# Autodesk Inventor assembly: Montagem peças superiores
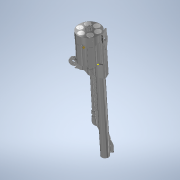
[picture p0: Inventor's stored thumbnail of the model, 180x180]
Saved by Autodesk Inventor 2021 (Build 250183000, 183)
## iProperties
Created: 2020-11-29
Part Number: Montagem peças superiores
Document SubType Name: Assembly
Designer: Bruno
Author: Bruno
## Documents named in this file (8)
- C:\Users\Bruno\Documents\Quadirmestre Suplementar\Projeto Assistido por Computador\Novas peças revólver\Montagem peças superiores.iam
- C:\Users\Bruno\Documents\Quadirmestre Suplementar\Projeto Assistido por Computador\Novas peças revólver\Cano do revólver.ipt
- C:\Users\Bruno\Documents\Quadirmestre Suplementar\Projeto Assistido por Computador\Novas peças revólver\Peça 15.ipt
- C:\Users\Bruno\Documents\Quadirmestre Suplementar\Projeto Assistido por Computador\Novas peças revólver\Peça 16.ipt
- C:\Users\Bruno\Documents\Quadirmestre Suplementar\Projeto Assistido por Computador\Novas peças revólver\Peça 17.ipt
- C:\Users\Bruno\Documents\Quadirmestre Suplementar\Projeto Assistido por Computador\Novas peças revólver\Baril do revólver.ipt
- C:\Users\Bruno\Documents\Quadirmestre Suplementar\Projeto Assistido por Computador\Novas peças revólver\Peça 18.ipt
- C:\Users\Bruno\Documents\Quadirmestre Suplementar\Projeto Assistido por Computador\Novas peças revólver\Bala do revólver.ipt
## Components (12 placed, 6 different names)
1. Cano do revólver:1 — Coincidente:1, Coincidente:2, Coincidente:4, Rotativa:1
2. Peça 15:1 — Coincidente:1, Coincidente:2, Coincidente:3
3. Peça 16:1 — Coincidente:3, Coincidente:4
4. Baril do revólver:1 — Coincidente:5, Rotativa:2, Coincidente:6
5. Baril do revólver:2 — Rotativa:1, Coincidente:5, Rotativa:2, Coincidente:7, Coincidente:8, Coincidente:9, Coincidente:10, Coincidente:11, Coincidente:12, Coincidente:13, Coincidente:14, Coincidente:15, Coincidente:16, Coincidente:17, Coincidente:18, Coincidente:19
6. Peça 18:1 — Coincidente:6, Coincidente:7
7. Bala do revólver:1 — Coincidente:10, Coincidente:11
8. Bala do revólver:2 — Coincidente:8, Coincidente:9
9. Bala do revólver:3 — Coincidente:14, Coincidente:15
10. Bala do revólver:4 — Coincidente:16, Coincidente:17
11. Bala do revólver:5 — Coincidente:18, Coincidente:19
12. Bala do revólver:6 — Coincidente:12, Coincidente:13
## Relationships (21: Mate 19, RevoluteJoint 2)
- Coincidente:1 [Mate]: Cano do revólver:1 ↔ Peça 15:1
- Coincidente:2 [Mate]: Cano do revólver:1 ↔ Peça 15:1
- Coincidente:3 [Mate] (18.18 mm): Peça 15:1 ↔ Peça 16:1
- Coincidente:4 [Mate] (0.056 mm): Cano do revólver:1 ↔ Peça 16:1
- Rotativa:1 [RevoluteJoint] (0.5 mm): Cano do revólver:1 ↔ Baril do revólver:2
- Coincidente:5 [Mate]: Baril do revólver:1 ↔ Baril do revólver:2
- Rotativa:2 [RevoluteJoint] (1.6 mm): Baril do revólver:1 ↔ Baril do revólver:2
- Coincidente:6 [Mate]: Baril do revólver:1 ↔ Peça 18:1
- Coincidente:7 [Mate]: Baril do revólver:2 ↔ Peça 18:1
- Coincidente:8 [Mate]: Baril do revólver:2 ↔ Bala do revólver:2
- Coincidente:9 [Mate]: Baril do revólver:2 ↔ Bala do revólver:2
- Coincidente:10 [Mate]: Baril do revólver:2 ↔ Bala do revólver:1
- Coincidente:11 [Mate]: Baril do revólver:2 ↔ Bala do revólver:1
- Coincidente:12 [Mate]: Baril do revólver:2 ↔ Bala do revólver:6
- Coincidente:13 [Mate]: Baril do revólver:2 ↔ Bala do revólver:6
- Coincidente:14 [Mate]: Baril do revólver:2 ↔ Bala do revólver:3
- Coincidente:15 [Mate]: Baril do revólver:2 ↔ Bala do revólver:3
- Coincidente:16 [Mate]: Baril do revólver:2 ↔ Bala do revólver:4
- Coincidente:17 [Mate]: Baril do revólver:2 ↔ Bala do revólver:4
- Coincidente:18 [Mate]: Baril do revólver:2 ↔ Bala do revólver:5
- Coincidente:19 [Mate]: Baril do revólver:2 ↔ Bala do revólver:5
